# Autodesk Inventor assembly: top gripper
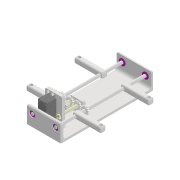
[picture p0: Inventor's stored thumbnail of the model, 180x180]
Saved by Autodesk Inventor 2020 (Build 240168000, 168)
## iProperties
Created: 2019-10-20
Part Number: top gripper
Document SubType Name: Assembly
Designer: ball
Author: ball
## Documents named in this file (11)
- C:\FTC\FTC8863CAD\2019 Robot\Collection\top gripper.iam
- C:\FTC\FTC8863CAD\RevRobotics\REV-41-1097.iam
- C:\FTC\FTC8863CAD\2019 Robot\Collection\Top grip collecter grip.ipt
- C:\FTC\FTC8863CAD\Actobotics\535 parts\535198.ipt
- C:\FTC\FTC8863CAD\Actobotics\634 parts\634088.ipt
- C:\FTC\FTC8863CAD\Actobotics\525 parts\525150 assembly.ipt
- C:\FTC\FTC8863CAD\Actobotics\634 parts\634058.ipt
- C:\FTC\FTC8863CAD\Actobotics\535 parts\535042.ipt
- C:\FTC\FTC8863CAD\Actobotics\634 parts\634068.ipt
- C:\FTC\FTC8863CAD\2019 Robot\Collection\Spur Gear 15T 24P 625c-c.ipt
- C:\FTC\FTC8863CAD\2019 Robot\Collection\Carrier arm.ipt
## Components (22 placed, 10 different names)
1. REV-41-1097:1 [sub-assembly] — Mate:3, Mate:14, Mate:15, Flush:12, Mate:29, Mate:30
2. Top grip collecter grip:1 — Mate:3, Mate:4, Mate:5, Mate:6, Mate:7, Mate:8, Mate:9, Mate:10, Mate:11, Flush:1, Flush:2, Mate:16, Mate:17, Mate:18, Mate:29, Mate:30, Mate:36, Mate:38, Mate:40, Mate:42
3. 535198:1 — Mate:4, Mate:5
4. 535198:2 — Mate:8, Mate:9, Mate:12
5. 535198:3 — Mate:6, Mate:7
6. 535198:4 — Mate:10, Mate:11, Mate:13
7. 634088:1 — Mate:13, Flush:2, Mate:33, Mate:35, Mate:37
8. 634088:2 — Mate:12, Flush:1, Mate:34, Mate:39, Mate:41
9. 525150 assembly:1 — Mate:14, Mate:15
10. 634058:2 — Mate:23, Flush:5, Flush:6, Flush:7, Mate:24, Mate:31
11. 535042:1 — Mate:23, Flush:5
12. 634068:1 — Flush:6, Flush:7, Mate:24, Mate:25, Flush:8, Mate:32
13. 535042:2 — Mate:25, Flush:8
14. 535042:3 — Flush:12
15. Spur Gear1:1 — Mate:34, Flush:15
16. Spur Gear1:2 — Mate:33, Flush:14
17. Spur Gear1:3 — Mate:32, Flush:13, Flush:14
18. Spur Gear1:4 — Mate:31, Flush:13, Flush:15
19. Carrier arm:1 — Mate:35, Mate:36
20. Carrier arm:2 — Mate:37, Mate:38
21. Carrier arm:3 — Mate:39, Mate:40
22. Carrier arm:4 — Mate:41, Mate:42
## Relationships (45: Mate 35, Flush 10)
- Mate:3 (8.4836 mm): REV-41-1097:1 ↔ Top grip collecter grip:1
- Mate:4: Top grip collecter grip:1 ↔ 535198:1
- Mate:5: Top grip collecter grip:1 ↔ 535198:1
- Mate:6: Top grip collecter grip:1 ↔ 535198:3
- Mate:7: Top grip collecter grip:1 ↔ 535198:3
- Mate:8: Top grip collecter grip:1 ↔ 535198:2
- Mate:9: Top grip collecter grip:1 ↔ 535198:2
- Mate:10: Top grip collecter grip:1 ↔ 535198:4
- Mate:11: Top grip collecter grip:1 ↔ 535198:4
- Mate:12: 535198:2 ↔ 634088:2
- Mate:13: 535198:4 ↔ 634088:1
- Flush:1: Top grip collecter grip:1 ↔ 634088:2
- Flush:2: Top grip collecter grip:1 ↔ 634088:1
- Mate:14: REV-41-1097:1 ↔ 525150 assembly:1
- Mate:15: REV-41-1097:1 ↔ 525150 assembly:1
- Mate:16: Top grip collecter grip:1
- Mate:17: Top grip collecter grip:1
- Mate:18: Top grip collecter grip:1
- [Mate]: 525150 assembly:1 ↔ 634058:2
- [Mate]: 525150 assembly:1 ↔ 634058:2
- Mate:23: 634058:2 ↔ 535042:1
- Flush:5: 634058:2 ↔ 535042:1
- Flush:6: 634058:2 ↔ 634068:1
- Flush:7: 634058:2 ↔ 634068:1
- Mate:24 (16.9418 mm): 634058:2 ↔ 634068:1
- Mate:25: 634068:1 ↔ 535042:2
- Flush:8: 634068:1 ↔ 535042:2
- Flush:12: REV-41-1097:1 ↔ 535042:3
- Mate:29 (2.5146 mm): REV-41-1097:1 ↔ Top grip collecter grip:1
- Mate:30: REV-41-1097:1 ↔ Top grip collecter grip:1
- Mate:31: 634058:2 ↔ Spur Gear1:4
- Mate:32: 634068:1 ↔ Spur Gear1:3
- Flush:13: Spur Gear1:3 ↔ Spur Gear1:4
- Mate:33: 634088:1 ↔ Spur Gear1:2
- Flush:14: Spur Gear1:2 ↔ Spur Gear1:3
- Mate:34: 634088:2 ↔ Spur Gear1:1
- Flush:15: Spur Gear1:1 ↔ Spur Gear1:4
- Mate:35: 634088:1 ↔ Carrier arm:1
- Mate:36 (38.1 mm): Top grip collecter grip:1 ↔ Carrier arm:1
- Mate:37: 634088:1 ↔ Carrier arm:2
- Mate:38 (38.1 mm): Top grip collecter grip:1 ↔ Carrier arm:2
- Mate:39: 634088:2 ↔ Carrier arm:3
- Mate:40 (38.1 mm): Top grip collecter grip:1 ↔ Carrier arm:3
- Mate:41: 634088:2 ↔ Carrier arm:4
- Mate:42 (38.1 mm): Top grip collecter grip:1 ↔ Carrier arm:4
